# Autodesk Inventor assembly: RoArm_cintura
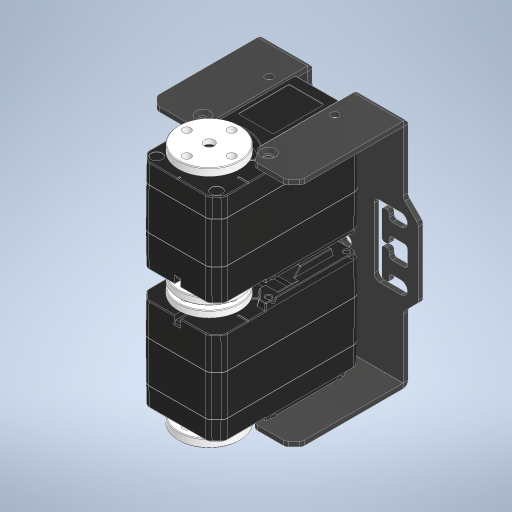
[picture p0: Inventor's stored thumbnail of the model, 512x512]
Saved by Autodesk Inventor 2024.4 (Build 284460000, 460)
## iProperties
Created: 2026-06-02
Part Number: RoArm_cintura
Document SubType Name: Assembly
Designer: epm01
Author: epm01
## Documents named in this file (3)
- D:\Archivos\2026-2\RoArm\inventor\RoArm_cintura.iam
- D:\Archivos\2026-2\RoArm\inventor\AL-BASE\AL-BASE\AL-BASE.ipt
- D:\Archivos\2026-2\RoArm\inventor\ST3215 v1\ST3215 v1\ST3215 v1.iam
## Components (3 placed, 2 different names)
1. AL-BASE:1 — Insert:1, Insert:2
2. ST3215 v1:1 [sub-assembly] — Insert:1, Flush:1
3. ST3215 v1:2 [sub-assembly] — Insert:2, Flush:1
## Relationships (3: Insert 2, Flush 1)
- Insert:1: AL-BASE:1 ↔ ST3215 v1:1
- Insert:2: AL-BASE:1 ↔ ST3215 v1:2
- Flush:1: ST3215 v1:1 ↔ ST3215 v1:2
